# Autodesk Inventor assembly: leg_tibea_ass
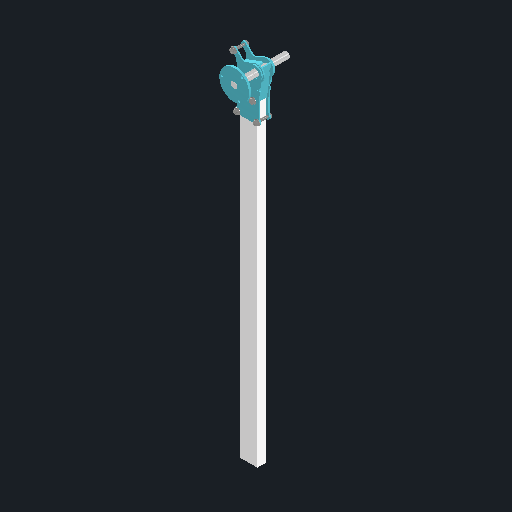
[picture p0: Inventor's stored thumbnail of the model, 512x512]
Saved by Autodesk Inventor 2026 (Build 300175000, 175)
## iProperties
Created: 2026-04-23
Part Number: leg_tibea_ass
Document SubType Name: Assembly
Designer: user
Mass: 1838.87 g
Surface Area: 2426.07 cm^2
Volume: 452.277 cm^3
Author: user
## Documents named in this file (19)
- C:\Users\user\vs_code_projects\ogonek-spider\physical-structure\cad\leg_tibea\leg_Right_tibea_ass.iam
- leg_Right_tibea_ass.iam
- C:\Users\user\vs_code_projects\ogonek-spider\physical-structure\cad\leg_tibea\tibea_profile.ipt
- C:\Users\user\vs_code_projects\ogonek-spider\physical-structure\cad\leg_tibea\tibea_outside_steel.ipt
- C:\Users\user\vs_code_projects\ogonek-spider\physical-structure\cad\leg_tibea\shaft_tibea.ipt
- C:\Users\user\vs_code_projects\ogonek-spider\physical-structure\cad\leg_tibea\tibea_vodilo_steel.ipt
- C:\Users\user\vs_code_projects\ogonek-spider\physical-structure\cad\leg_tibea\tibea_reinforcement_steel.ipt
- C:\Users\user\vs_code_projects\ogonek-spider\physical-structure\cad\leg_tibea\tibea_reinforcment2_steel.ipt
- C:\Users\user\vs_code_projects\ogonek-spider\physical-structure\cad\leg_tibea\tibea_ring_for_bearing_tibea.ipt
- C:\Users\user\Documents\Inventor\Content Center Files\R2026\ru-RU\Bolt 2 GOST 15591-70\Болт 2 M6×32 ГОСТ 15591-70.ipt
- C:\Users\user\Documents\Inventor\Content Center Files\R2026\ru-RU\Nut GOST R ISO 4161-2013\ГайкаM6-6H ГОСТ Р ISO 4161-2013.ipt
- C:\Users\user\vs_code_projects\ogonek-spider\physical-structure\cad\parametres.xlsx
- C:\Users\user\vs_code_projects\ogonek-spider\physical-structure\cad\leg_tibea\leg_Left_tibea_ass\AIP\FEA\fer4zszvk.fins
- C:\Users\user\vs_code_projects\ogonek-spider\physical-structure\cad\leg_tibea\leg_Left_tibea_ass\AIP\FEA\fer4zszvk.fsat
- C:\Users\user\vs_code_projects\ogonek-spider\physical-structure\cad\leg_tibea\leg_Left_tibea_ass\AIP\FEA\fer4zszvk.ftes
- C:\Users\user\vs_code_projects\ogonek-spider\physical-structure\cad\leg_tibea\leg_Left_tibea_ass\AIP\FEA\fer4zszvk.fwiz
- C:\Users\user\vs_code_projects\ogonek-spider\physical-structure\cad\leg_tibea\leg_Left_tibea_ass\AIP\FEA\fer4zszy8.fmsh
- C:\Users\user\vs_code_projects\ogonek-spider\physical-structure\cad\leg_tibea\leg_Left_tibea_ass\AIP\FEA\fer8dcvr4.fres
- C:\Users\user\vs_code_projects\ogonek-spider\physical-structure\cad\leg_tibea\leg_Right_tibea_ass\AIP\FEA\ff2ryorfk.fres
## Components (21 placed, 9 different names)
1. tibea_profile:1 — Жесткий:3, Жесткий:13, Совмещение:2
2. tibea_outside_steel:1 — Жесткий:3, Жесткий:16, Совмещение:16, Совмещение:18, Совмещение:20, Совмещение:22, Совмещение:24, Совмещение:26
3. tibea_outside_steel:2 — Жесткий:13, Совмещение:1, Жесткий:15, Жесткий:17, Совмещение:3, Совмещение:4, Совмещение:5, Совмещение:6, Совмещение:7, Совмещение:8, Совмещение:9, Совмещение:10, Совмещение:11, Совмещение:12, Совмещение:13, Совмещение:14, Совмещение:15, Совмещение:17, Совмещение:19, Совмещение:21, Совмещение:23, Совмещение:25
4. tibea_reinforcement_steel:2 — Совмещение:1, Касательность:1, Касательность:2, Совмещение:2
5. tibea_reinforcment2_steel:1 — Жесткий:17
6. tibea_ring_for_bearing_tibea:1 — Жесткий:15, Жесткий:11
7. tibea_ring_for_bearing_tibea:2 — Жесткий:16
8. tibea_vodilo_steel:1 — Жесткий:10
9. shaft_tibea:1 — Жесткий:10, Жесткий:11, Касательность:1, Касательность:2
10. Болт 2 ГОСТ 15591-70 M6×32:1 — Совмещение:3, Совмещение:4
11. Гайка ГОСТ Р ISO 4161-2013 M6:1 — Совмещение:15, Совмещение:16
12. Болт 2 ГОСТ 15591-70 M6×32:2 — Совмещение:5, Совмещение:6
13. Болт 2 ГОСТ 15591-70 M6×32:3 — Совмещение:7, Совмещение:8
14. Болт 2 ГОСТ 15591-70 M6×32:4 — Совмещение:9, Совмещение:10
15. Болт 2 ГОСТ 15591-70 M6×32:5 — Совмещение:11, Совмещение:12
16. Болт 2 ГОСТ 15591-70 M6×32:6 — Совмещение:13, Совмещение:14
17. Гайка ГОСТ Р ISO 4161-2013 M6:2 — Совмещение:17, Совмещение:18
18. Гайка ГОСТ Р ISO 4161-2013 M6:3 — Совмещение:19, Совмещение:20
19. Гайка ГОСТ Р ISO 4161-2013 M6:4 — Совмещение:21, Совмещение:22
20. Гайка ГОСТ Р ISO 4161-2013 M6:5 — Совмещение:23, Совмещение:24
21. Гайка ГОСТ Р ISO 4161-2013 M6:6 — Совмещение:25, Совмещение:26
## Relationships (35: Mate 26, WeldJoint 7, Tangent 2)
- Жесткий:3 [WeldJoint]: tibea_profile:1 ↔ tibea_outside_steel:1
- Жесткий:10 [WeldJoint] (-1 mm): tibea_vodilo_steel:1 ↔ shaft_tibea:1
- Жесткий:11 [WeldJoint] (43 mm): tibea_ring_for_bearing_tibea:1 ↔ shaft_tibea:1
- Жесткий:13 [WeldJoint]: tibea_profile:1 ↔ tibea_outside_steel:2
- Совмещение:1 [Mate]: tibea_outside_steel:2 ↔ tibea_reinforcement_steel:2
- Касательность:1 [Tangent]: tibea_reinforcement_steel:2 ↔ shaft_tibea:1
- Касательность:2 [Tangent]: tibea_reinforcement_steel:2 ↔ shaft_tibea:1
- Совмещение:2 [Mate]: tibea_profile:1 ↔ tibea_reinforcement_steel:2
- Жесткий:15 [WeldJoint]: tibea_outside_steel:2 ↔ tibea_ring_for_bearing_tibea:1
- Жесткий:16 [WeldJoint]: tibea_outside_steel:1 ↔ tibea_ring_for_bearing_tibea:2
- Жесткий:17 [WeldJoint]: tibea_outside_steel:2 ↔ tibea_reinforcment2_steel:1
- Совмещение:3 [Mate]: tibea_outside_steel:2 ↔ Болт 2 ГОСТ 15591-70 M6×32:1
- Совмещение:4 [Mate]: tibea_outside_steel:2 ↔ Болт 2 ГОСТ 15591-70 M6×32:1
- Совмещение:5 [Mate]: tibea_outside_steel:2 ↔ Болт 2 ГОСТ 15591-70 M6×32:2
- Совмещение:6 [Mate]: tibea_outside_steel:2 ↔ Болт 2 ГОСТ 15591-70 M6×32:2
- Совмещение:7 [Mate]: tibea_outside_steel:2 ↔ Болт 2 ГОСТ 15591-70 M6×32:3
- Совмещение:8 [Mate]: tibea_outside_steel:2 ↔ Болт 2 ГОСТ 15591-70 M6×32:3
- Совмещение:9 [Mate]: tibea_outside_steel:2 ↔ Болт 2 ГОСТ 15591-70 M6×32:4
- Совмещение:10 [Mate]: tibea_outside_steel:2 ↔ Болт 2 ГОСТ 15591-70 M6×32:4
- Совмещение:11 [Mate]: tibea_outside_steel:2 ↔ Болт 2 ГОСТ 15591-70 M6×32:5
- Совмещение:12 [Mate]: tibea_outside_steel:2 ↔ Болт 2 ГОСТ 15591-70 M6×32:5
- Совмещение:13 [Mate]: tibea_outside_steel:2 ↔ Болт 2 ГОСТ 15591-70 M6×32:6
- Совмещение:14 [Mate]: tibea_outside_steel:2 ↔ Болт 2 ГОСТ 15591-70 M6×32:6
- Совмещение:15 [Mate]: tibea_outside_steel:2 ↔ Гайка ГОСТ Р ISO 4161-2013 M6:1
- Совмещение:16 [Mate]: tibea_outside_steel:1 ↔ Гайка ГОСТ Р ISO 4161-2013 M6:1
- Совмещение:17 [Mate]: tibea_outside_steel:2 ↔ Гайка ГОСТ Р ISO 4161-2013 M6:2
- Совмещение:18 [Mate]: tibea_outside_steel:1 ↔ Гайка ГОСТ Р ISO 4161-2013 M6:2
- Совмещение:19 [Mate]: tibea_outside_steel:2 ↔ Гайка ГОСТ Р ISO 4161-2013 M6:3
- Совмещение:20 [Mate]: tibea_outside_steel:1 ↔ Гайка ГОСТ Р ISO 4161-2013 M6:3
- Совмещение:21 [Mate]: tibea_outside_steel:2 ↔ Гайка ГОСТ Р ISO 4161-2013 M6:4
- Совмещение:22 [Mate]: tibea_outside_steel:1 ↔ Гайка ГОСТ Р ISO 4161-2013 M6:4
- Совмещение:23 [Mate]: tibea_outside_steel:2 ↔ Гайка ГОСТ Р ISO 4161-2013 M6:5
- Совмещение:24 [Mate]: tibea_outside_steel:1 ↔ Гайка ГОСТ Р ISO 4161-2013 M6:5
- Совмещение:25 [Mate]: tibea_outside_steel:2 ↔ Гайка ГОСТ Р ISO 4161-2013 M6:6
- Совмещение:26 [Mate]: tibea_outside_steel:1 ↔ Гайка ГОСТ Р ISO 4161-2013 M6:6
## Named parameters: tolerance_plazma = 0.1 mm, thickness_steel = 3 mm, d_main_screw_holes = 6.1 mm, d_main_shaft = 15 mm, thickness_profile_tibea = 3 mm, width_profile_tibea = 20 mm, hight_profile_tibea = 40 mm, length_profile_tibia = 800 mm, length_thorn_tibia = 400 mm, width_shaft_shift = 35 mm, length_profile_femur = 350 mm, thickness_profile_femur = 3 mm, width_profile_femur = 50 mm, hight_shaft_shift = 37 mm, hight_profile_femur = 50 mm, width_flattened_surface = 12 mm, sa_0 = 600000, length_coxa = 100 mm, hight_coxa = 40 mm, width_coxa = 80 mm, width_body_l1 = 100 mm, width_body_l2 = 150 mm, width_body_l3 = 120 mm, offset_body_l12 = 60 mm, offset_body_l12_1 = 200 mm, offset_body_l23 = 200 mm, hight_ground_clearance = 500 mm, sa_1 = 0, sa_2 = -50000, sa_3 = 0
note: some values were not read from the file. Shown as the stored number, unit unknown: "sa_0", "sa_1", "sa_2", "sa_3".
